# Autodesk Inventor assembly: Battery Rack Assembly
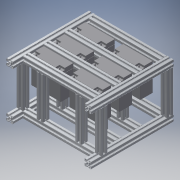
[picture p0: Inventor's stored thumbnail of the model, 180x180]
Saved by Autodesk Inventor 2019.4 (Build 234330000, 330)
## iProperties
Created: 2020-02-27
Part Number: Battery Rack Assembly
Document SubType Name: Assembly
Designer: admin
Author: admin
## Documents named in this file (5)
- C:\Users\admin\Desktop\FRC 2020 Engineering\GitHub\7738-2020\Pit Station Designs\battery rack\Battery Rack Assembly.iam
- C:\Users\admin\Desktop\FRC 2020 Engineering\GitHub\7738-2020\CAD\Battery.ipt
- C:\Users\admin\Desktop\FRC 2020 Engineering\GitHub\7738-2020\Pit Station Designs\battery rack\Extrusion 1.ipt
- C:\Users\admin\Desktop\FRC 2020 Engineering\GitHub\7738-2020\Pit Station Designs\battery rack\Extrusion 2.ipt
- C:\Users\admin\Desktop\FRC 2020 Engineering\GitHub\7738-2020\Pit Station Designs\battery rack\Extrusion 3.ipt
## Components (28 placed, 4 different names)
1. Battery:1 — Flush:1, Mate:1, Flush:5, Flush:8, Flush:11, Mate:6
2. Battery:2 — Flush:3, Mate:4, Flush:5, Flush:8, Flush:10, Mate:17
3. Battery:3 — Flush:3, Flush:4, Mate:3, Mate:4, Flush:7, Flush:9, Flush:10, Mate:16
4. Battery:4 — Flush:1, Flush:2, Mate:1, Mate:2, Flush:7
5. Battery:5 — Flush:4, Mate:3, Mate:5, Flush:6, Flush:9, Mate:13
6. Battery:6 — Flush:2, Mate:2, Mate:5, Flush:6, Flush:14
7. Extrusion 1:1 — Mate:7, Mate:10, Flush:15, Flush:32, Flush:33, Mate:22, Mate:23, Flush:34
8. Extrusion 1:2 — Mate:8, Flush:13, Flush:14, Flush:16, Mate:11, Flush:21, Flush:22
9. Extrusion 1:3 — Flush:12, Mate:9, Mate:10, Flush:15, Mate:12, Flush:17, Flush:18, Mate:14, Mate:15, Flush:19, Flush:20, Flush:23
10. Extrusion 1:4 — Flush:16, Mate:11, Flush:21, Flush:24, Mate:18, Mate:19, Mate:20, Mate:21, Flush:26, Flush:27, Flush:28, Flush:29, Mate:24, Mate:25, Flush:36, Flush:37
11. Extrusion 2:1 — Mate:7, Mate:8, Flush:12, Flush:13, Mate:9, Mate:13, Flush:23, Flush:25, Flush:39
12. Extrusion 2:2 — Mate:12, Flush:17, Mate:16, Flush:30
13. Extrusion 2:3 — Mate:15, Flush:19, Flush:20, Flush:22, Flush:38
14. Extrusion 2:4 — Flush:18, Mate:14, Mate:17, Flush:31
15. Extrusion 2:5 — Flush:24, Mate:18, Flush:25, Flush:35, Mate:28, Mate:29, Flush:42, Flush:43
16. Extrusion 2:6 — Mate:19, Flush:29, Flush:30, Mate:26, Mate:30, Flush:41, Flush:44
17. Extrusion 2:7 — Mate:20, Flush:28, Flush:31, Mate:27, Mate:31, Flush:40, Flush:45
18. Extrusion 2:8 — Mate:21, Flush:26, Flush:27
19. Extrusion 3:1 — Flush:32, Mate:22, Flush:35
20. Extrusion 3:2 — Mate:24, Flush:37, Flush:38
21. Extrusion 3:3 — Mate:25, Flush:36, Flush:39
22. Extrusion 3:4 — Flush:33, Mate:23, Flush:34
23. Extrusion 3:5 — Mate:26, Flush:44
24. Extrusion 3:6 — Mate:29, Flush:42
25. Extrusion 3:7 — Mate:27, Flush:45
26. Extrusion 3:8 — Mate:30, Flush:41
27. Extrusion 3:9 — Mate:28, Flush:43
28. Extrusion 3:10 — Mate:31, Flush:40
## Relationships (76: Flush 45, Mate 31)
- Flush:1: Battery:1 ↔ Battery:4
- Flush:2: Battery:4 ↔ Battery:6
- Flush:3: Battery:2 ↔ Battery:3
- Flush:4: Battery:3 ↔ Battery:5
- Mate:1 (50 mm): Battery:1 ↔ Battery:4
- Mate:2 (50 mm): Battery:4 ↔ Battery:6
- Mate:3 (50 mm): Battery:3 ↔ Battery:5
- Mate:4 (50 mm): Battery:2 ↔ Battery:3
- Mate:5 (50 mm): Battery:5 ↔ Battery:6
- Flush:5: Battery:1 ↔ Battery:2
- Flush:6: Battery:5 ↔ Battery:6
- Flush:7: Battery:3 ↔ Battery:4
- Flush:8: Battery:1 ↔ Battery:2
- Flush:9: Battery:3 ↔ Battery:5
- Flush:10: Battery:2 ↔ Battery:3
- Flush:11: Battery:1
- Mate:6: Battery:1
- Mate:7: Extrusion 1:1 ↔ Extrusion 2:1
- Mate:8: Extrusion 1:2 ↔ Extrusion 2:1
- Flush:12: Extrusion 1:3 ↔ Extrusion 2:1
- Flush:13: Extrusion 1:2 ↔ Extrusion 2:1
- Flush:14: Battery:6 ↔ Extrusion 1:2
- Mate:9: Extrusion 1:3 ↔ Extrusion 2:1
- Mate:10 (250 mm): Extrusion 1:1 ↔ Extrusion 1:3
- Flush:15: Extrusion 1:1 ↔ Extrusion 1:3
- Flush:16: Extrusion 1:2 ↔ Extrusion 1:4
- Mate:11 (250 mm): Extrusion 1:2 ↔ Extrusion 1:4
- Mate:12: Extrusion 1:3 ↔ Extrusion 2:2
- Flush:17: Extrusion 1:3 ↔ Extrusion 2:2
- Mate:13: Battery:5 ↔ Extrusion 2:1
- Flush:18: Extrusion 1:3 ↔ Extrusion 2:4
- Mate:14: Extrusion 1:3 ↔ Extrusion 2:4
- Mate:15: Extrusion 1:3 ↔ Extrusion 2:3
- Mate:16: Battery:3 ↔ Extrusion 2:2
- Mate:17: Battery:2 ↔ Extrusion 2:4
- Flush:19: Extrusion 1:3 ↔ Extrusion 2:3
- Flush:20: Extrusion 1:3 ↔ Extrusion 2:3
- Flush:21: Extrusion 1:2 ↔ Extrusion 1:4
- Flush:22: Extrusion 1:2 ↔ Extrusion 2:3
- Flush:23 (-60 mm): Extrusion 1:3 ↔ Extrusion 2:1
- Flush:24: Extrusion 1:4 ↔ Extrusion 2:5
- Mate:18: Extrusion 1:4 ↔ Extrusion 2:5
- Flush:25: Extrusion 2:1 ↔ Extrusion 2:5
- Mate:19: Extrusion 1:4 ↔ Extrusion 2:6
- Mate:20: Extrusion 1:4 ↔ Extrusion 2:7
- Mate:21: Extrusion 1:4 ↔ Extrusion 2:8
- Flush:26: Extrusion 1:4 ↔ Extrusion 2:8
- Flush:27: Extrusion 1:4 ↔ Extrusion 2:8
- Flush:28: Extrusion 1:4 ↔ Extrusion 2:7
- Flush:29: Extrusion 1:4 ↔ Extrusion 2:6
- Flush:30: Extrusion 2:2 ↔ Extrusion 2:6
- Flush:31: Extrusion 2:4 ↔ Extrusion 2:7
- Flush:32: Extrusion 1:1 ↔ Extrusion 3:1
- Flush:33: Extrusion 1:1 ↔ Extrusion 3:4
- Mate:22: Extrusion 1:1 ↔ Extrusion 3:1
- Mate:23: Extrusion 1:1 ↔ Extrusion 3:4
- Flush:34: Extrusion 1:1 ↔ Extrusion 3:4
- Flush:35: Extrusion 2:5 ↔ Extrusion 3:1
- Mate:24: Extrusion 1:4 ↔ Extrusion 3:2
- Mate:25: Extrusion 1:4 ↔ Extrusion 3:3
- Flush:36: Extrusion 1:4 ↔ Extrusion 3:3
- Flush:37: Extrusion 1:4 ↔ Extrusion 3:2
- Flush:38: Extrusion 2:3 ↔ Extrusion 3:2
- Flush:39: Extrusion 2:1 ↔ Extrusion 3:3
- Mate:26: Extrusion 2:6 ↔ Extrusion 3:5
- Mate:27: Extrusion 2:7 ↔ Extrusion 3:7
- Mate:28: Extrusion 2:5 ↔ Extrusion 3:9
- Mate:29: Extrusion 2:5 ↔ Extrusion 3:6
- Mate:30: Extrusion 2:6 ↔ Extrusion 3:8
- Mate:31: Extrusion 2:7 ↔ Extrusion 3:10
- Flush:40: Extrusion 2:7 ↔ Extrusion 3:10
- Flush:41: Extrusion 2:6 ↔ Extrusion 3:8
- Flush:42: Extrusion 2:5 ↔ Extrusion 3:6
- Flush:43: Extrusion 2:5 ↔ Extrusion 3:9
- Flush:44: Extrusion 2:6 ↔ Extrusion 3:5
- Flush:45: Extrusion 2:7 ↔ Extrusion 3:7
